# Autodesk Inventor assembly: bellows_latest
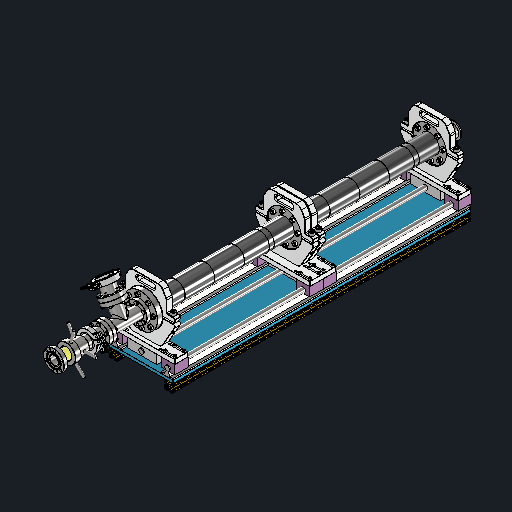
[picture p0: Inventor's stored thumbnail of the model, 512x512]
Saved by Autodesk Inventor 2027.1 (Build 311270010, 270A)
## iProperties
Created: 2026-06-04
Part Number: bellows_latest
Document SubType Name: Assembly
Designer: shusu
Author: shusu
## Documents named in this file (20)
- C:\Users\queezz\Dropbox\Drawings\pihti-cad\bellows-probe\sliding-assembly.iam
- C:\Users\queezz\Dropbox\Drawings\pihti-cad\bellows-probe\rail bwllows probe.ipt
- C:\Users\queezz\Dropbox\Drawings\pihti-cad\bellows-probe\Al-profile-30x30-L1000.ipt
- C:\Users\queezz\Dropbox\Drawings\pihti-cad\ContentCenter\Aluminium-profiles\Al-profile-30x30.ipt
- C:\Users\queezz\Dropbox\Drawings\pihti-cad\bellows-probe\base-plate-for-bellows.ipt
- C:\Users\queezz\Dropbox\Drawings\pihti-cad\ContentCenter\Fastners\M6x16-SHCS.ipt
- C:\Users\queezz\Dropbox\Drawings\pihti-cad\ContentCenter\CF-KF-adapters\ICF70_to_KF40.ipt
- C:\Users\queezz\Dropbox\Drawings\pihti-cad\bellows-probe\CF114-CF70-zero-length-adappter.ipt
- C:\Users\queezz\Dropbox\Drawings\pihti-cad\bellows-probe\M16-lead-screw.ipt
- C:\Users\queezz\Dropbox\Drawings\pihti-cad\bellows-probe\lead-screw-nut-preview.ipt
- C:\Users\queezz\Dropbox\Drawings\pihti-cad\bellows-probe\two-section-bellows-on-bearings.iam
- C:\Users\queezz\Dropbox\Drawings\pihti-cad\ContentCenter\Fastners\m8-nut.ipt
- C:\Users\queezz\Dropbox\Drawings\pihti-cad\ContentCenter\Fastners\M8x45-HexCS.ipt
- C:\Users\queezz\Dropbox\Drawings\pihti-cad\bellows-probe\mizuno-pipe.iam
- C:\Users\queezz\Dropbox\Drawings\pihti-cad\Plasma Vessel\pipe-o-ring-gauge-port-assembly.iam
- C:\Users\queezz\Dropbox\Drawings\pihti-cad\ContentCenter\CF-parts\CF-70-Tee.ipt
- C:\Users\queezz\Dropbox\Drawings\pihti-cad\ContentCenter\Fastners\M6x25-HexCS.ipt
- C:\Users\queezz\Dropbox\Drawings\pihti-cad\ContentCenter\Fastners\M6x35-HexCS.ipt
- C:\Users\queezz\Dropbox\Drawings\pihti-cad\ContentCenter\Fastners\M6-nut.ipt
- C:\Users\queezz\Dropbox\Drawings\pihti-cad\ContentCenter\NW\NW40_clamp.ipt
## Components (82 placed, 45 different names)
1. rail:1 — Mate:9, Flush:22, Mate:30
2. rail:2 — Mate:9, Mate:16, Flush:12, Flush:20
3. Al-profile-30x30-L1000:1 — Mate:18, Flush:13, Flush:16
4. Al-profile-30x30-L1000:2 — Mate:17, Flush:14, Flush:15
5. base-plate-for-bellows:1 — Mate:16, Flush:11, Flush:12, Mate:17, Mate:18, Flush:13, Flush:14, Flush:15, Flush:16, Flush:22, Mate:30, Flush:24
6. ICF70_to_KF40:1 — Rotational:6, Mate:31
7. CF114-CF70-zero-length-adappter:1 — Rotational:6, Rear flange bolt 1 - rigid, Rear flange bolt 2 - rigid, Rear flange bolt 3 - rigid, Rear flange bolt 4 - rigid, Rear flange bolt 5 - rigid, Rear flange bolt 6 - rigid, Rear flange bolt 7 - rigid, Rear flange bolt 8 - rigid
8. M16-lead-screw:1 — Mate:26, Flush:20
9. lead-screw-nut-preview:1 — Mate:26, Rigid:25
10. lead-screw-nut-preview:2
11. lead-screw-nut-preview:4
12. two-section-bellows-on-bearings:1 [sub-assembly] — Rigid:25, Rigid:26, Front flange nut 1 - rigid, Rear flange nut 1 - rigid, Front flange nut 2 - rigid, Front flange nut 3 - rigid, Front flange nut 4 - rigid, Front flange nut 5 - rigid, Front flange nut 6 - rigid, Front flange nut 7 - rigid, Front flange nut 8 - rigid, Rear flange nut 2 - rigid, Rear flange nut 3 - rigid, Rear flange nut 4 - rigid, Rear flange nut 5 - rigid, Rear flange nut 6 - rigid, Rear flange nut 7 - rigid, Rear flange nut 8 - rigid, Flush:24
13. CF114-CF70-zero-length-adappter:2 — Rigid:26, Front flange bolt 1 - rigid, Front flange bolt 2 - rigid, Front flange bolt 3 - rigid, Front flange bolt 4 - rigid, Front flange bolt 5 - rigid, Front flange bolt 6 - rigid, Front flange bolt 7 - rigid, Front flange bolt 8 - rigid, Rigid:60, Flush:23, Bypass tee to bellows adapter - rigid
14. mizuno-pipe:1 [sub-assembly] — Mate:31, Flush:23
15. pipe-o-ring-gauge-port-assembly:1 [sub-assembly] — Rigid:60, Gauge port to bypass tee - rigid, Bypass gauge nut 1 - rigid, Bypass gauge nut 2 - rigid, Bypass gauge nut 3 - rigid, Bypass gauge nut 4 - rigid, Bypass gauge nut 5 - rigid, Bypass gauge nut 6 - rigid
16. CF-70-Tee:1 — Bypass tee to bellows adapter - rigid, Gauge port to bypass tee - rigid, Bypass bellows bolt 1 - rigid, Bypass bellows bolt 2 - rigid, Bypass bellows bolt 3 - rigid, Bypass bellows bolt 4 - rigid, Bypass bellows bolt 5 - rigid, Bypass bellows bolt 6 - rigid, Bypass gauge bolt 1 - rigid, Bypass gauge bolt 2 - rigid, Bypass gauge bolt 3 - rigid, Bypass gauge bolt 4 - rigid, Bypass gauge bolt 5 - rigid, Bypass gauge bolt 6 - rigid, Rigid:81, Bypass branch bolt 1 - rigid, Bypass branch bolt 2 - rigid, Bypass branch bolt 3 - rigid, Bypass branch bolt 4 - rigid, Bypass branch bolt 5 - rigid, Bypass branch bolt 6 - rigid
17. ICF70_to_KF40:2 — Rigid:81, Bypass branch nut 1 - rigid, Bypass branch nut 2 - rigid, Bypass branch nut 3 - rigid, Bypass branch nut 4 - rigid, Bypass branch nut 5 - rigid, Bypass branch nut 6 - rigid, Bypass KF40 clamp to adapter - rigid
18. Bypass branch bolt 1 — Bypass branch bolt 1 - rigid
19. Bypass branch nut 1 — Bypass branch nut 1 - rigid
20. Bypass branch bolt 2 — Bypass branch bolt 2 - rigid
21. Bypass branch nut 2 — Bypass branch nut 2 - rigid
22. Bypass branch bolt 3 — Bypass branch bolt 3 - rigid
23. Bypass branch nut 3 — Bypass branch nut 3 - rigid
24. Bypass branch bolt 4 — Bypass branch bolt 4 - rigid
25. Bypass branch nut 4 — Bypass branch nut 4 - rigid
26. Bypass branch bolt 5 — Bypass branch bolt 5 - rigid
27. Bypass branch nut 5 — Bypass branch nut 5 - rigid
28. Bypass branch bolt 6 — Bypass branch bolt 6 - rigid
29. Bypass branch nut 6 — Bypass branch nut 6 - rigid
30. Bypass branch KF40 clamp:1 — Bypass KF40 clamp to adapter - rigid
31. Bypass bellows bolt 1 — Bypass bellows bolt 1 - rigid
32. Bypass bellows bolt 2 — Bypass bellows bolt 2 - rigid
33. Bypass bellows bolt 3 — Bypass bellows bolt 3 - rigid
34. Bypass bellows bolt 4 — Bypass bellows bolt 4 - rigid
35. Bypass bellows bolt 5 — Bypass bellows bolt 5 - rigid
36. Bypass bellows bolt 6 — Bypass bellows bolt 6 - rigid
37. Bypass gauge bolt 1 — Bypass gauge bolt 1 - rigid
38. Bypass gauge nut 1 — Bypass gauge nut 1 - rigid
39. Bypass gauge bolt 2 — Bypass gauge bolt 2 - rigid
40. Bypass gauge nut 2 — Bypass gauge nut 2 - rigid
41. Bypass gauge bolt 3 — Bypass gauge bolt 3 - rigid
42. Bypass gauge nut 3 — Bypass gauge nut 3 - rigid
43. Bypass gauge bolt 4 — Bypass gauge bolt 4 - rigid
44. Bypass gauge nut 4 — Bypass gauge nut 4 - rigid
45. Bypass gauge bolt 5 — Bypass gauge bolt 5 - rigid
46. Bypass gauge nut 5 — Bypass gauge nut 5 - rigid
47. Bypass gauge bolt 6 — Bypass gauge bolt 6 - rigid
48. Bypass gauge nut 6 — Bypass gauge nut 6 - rigid
49. AS 1112 (2) - Metric M8  Type 5:1 — Front flange nut 1 - rigid
50. AS 1427 - Metric M8 x 45:1 — Front flange bolt 1 - rigid
51. AS 1427 - Metric M8 x 45:2 — Rear flange bolt 1 - rigid
52. AS 1112 (2) - Metric M8  Type 5:2 — Rear flange nut 1 - rigid
53. AS 1427 - Metric M8 x 45:3 — Front flange bolt 2 - rigid
54. AS 1427 - Metric M8 x 45:4 — Front flange bolt 3 - rigid
55. AS 1427 - Metric M8 x 45:5 — Front flange bolt 4 - rigid
56. AS 1427 - Metric M8 x 45:6 — Front flange bolt 5 - rigid
57. AS 1427 - Metric M8 x 45:7 — Front flange bolt 6 - rigid
58. AS 1427 - Metric M8 x 45:8 — Front flange bolt 7 - rigid
59. AS 1427 - Metric M8 x 45:9 — Front flange bolt 8 - rigid
60. AS 1427 - Metric M8 x 45:10 — Rear flange bolt 2 - rigid
61. AS 1427 - Metric M8 x 45:11 — Rear flange bolt 3 - rigid
62. AS 1427 - Metric M8 x 45:12 — Rear flange bolt 4 - rigid
63. AS 1427 - Metric M8 x 45:13 — Rear flange bolt 5 - rigid
64. AS 1427 - Metric M8 x 45:14 — Rear flange bolt 6 - rigid
65. AS 1427 - Metric M8 x 45:15 — Rear flange bolt 7 - rigid
66. AS 1427 - Metric M8 x 45:16 — Rear flange bolt 8 - rigid
67. AS 1112 (2) - Metric M8  Type 5:3 — Front flange nut 2 - rigid
68. AS 1112 (2) - Metric M8  Type 5:4 — Front flange nut 3 - rigid
69. AS 1112 (2) - Metric M8  Type 5:5 — Front flange nut 4 - rigid
70. AS 1112 (2) - Metric M8  Type 5:6 — Front flange nut 5 - rigid
71. AS 1112 (2) - Metric M8  Type 5:7 — Front flange nut 6 - rigid
72. AS 1112 (2) - Metric M8  Type 5:8 — Front flange nut 7 - rigid
73. AS 1112 (2) - Metric M8  Type 5:9 — Front flange nut 8 - rigid
74. AS 1112 (2) - Metric M8  Type 5:10 — Rear flange nut 2 - rigid
75. AS 1112 (2) - Metric M8  Type 5:11 — Rear flange nut 3 - rigid
76. AS 1112 (2) - Metric M8  Type 5:12 — Rear flange nut 4 - rigid
77. AS 1112 (2) - Metric M8  Type 5:13 — Rear flange nut 5 - rigid
78. AS 1112 (2) - Metric M8  Type 5:14 — Rear flange nut 6 - rigid
79. AS 1112 (2) - Metric M8  Type 5:15 — Rear flange nut 7 - rigid
80. AS 1112 (2) - Metric M8  Type 5:16 — Rear flange nut 8 - rigid
81. JIS B 1176 - Metric M6 x 16:3
82. JIS B 1176 - Metric M6 x 16:4
## Relationships (100: WeldJoint 74, Mate 15, Flush 10, RevoluteJoint 1)
- [Mate]: rail:1 ↔ two-section-bellows-on-bearings:1
- [Mate]: rail:2 ↔ two-section-bellows-on-bearings:1
- [Mate]: rail:2 ↔ two-section-bellows-on-bearings:1
- [Mate]: rail:1 ↔ two-section-bellows-on-bearings:1
- Mate:9 (175 mm): rail:1 ↔ rail:2
- [Mate]: two-section-bellows-on-bearings:1
- [Mate]: two-section-bellows-on-bearings:1
- Mate:16: rail:2 ↔ base-plate-for-bellows:1
- Flush:11: base-plate-for-bellows:1
- Flush:12: rail:2 ↔ base-plate-for-bellows:1
- Mate:17: Al-profile-30x30-L1000:2 ↔ base-plate-for-bellows:1
- Mate:18: Al-profile-30x30-L1000:1 ↔ base-plate-for-bellows:1
- Flush:13: Al-profile-30x30-L1000:1 ↔ base-plate-for-bellows:1
- Flush:14: Al-profile-30x30-L1000:2 ↔ base-plate-for-bellows:1
- Flush:15: Al-profile-30x30-L1000:2 ↔ base-plate-for-bellows:1
- Flush:16: Al-profile-30x30-L1000:1 ↔ base-plate-for-bellows:1
- [WeldJoint]: two-section-bellows-on-bearings:1 ↔ JIS B 1176 - Metric M6 x 16:3
- [WeldJoint]: two-section-bellows-on-bearings:1 ↔ JIS B 1176 - Metric M6 x 16:4
- [WeldJoint]: CF114-CF70-zero-length-adappter:1 ↔ two-section-bellows-on-bearings:1
- Rotational:6 [RevoluteJoint]: ICF70_to_KF40:1 ↔ CF114-CF70-zero-length-adappter:1
- Mate:26: M16-lead-screw:1 ↔ lead-screw-nut-preview:1
- Flush:20: rail:2 ↔ M16-lead-screw:1
- [WeldJoint]: lead-screw-nut-preview:2 ↔ two-section-bellows-on-bearings:1
- [Mate]: rail:1 ↔ two-section-bellows-on-bearings:1
- [Mate]: rail:2 ↔ two-section-bellows-on-bearings:1
- [WeldJoint]: lead-screw-nut-preview:4 ↔ two-section-bellows-on-bearings:1
- Rigid:25 [WeldJoint]: lead-screw-nut-preview:1 ↔ two-section-bellows-on-bearings:1
- Rigid:26 [WeldJoint]: two-section-bellows-on-bearings:1 ↔ CF114-CF70-zero-length-adappter:2
- Front flange nut 1 - rigid [WeldJoint]: two-section-bellows-on-bearings:1 ↔ AS 1112 (2) - Metric M8  Type 5:1
- Front flange bolt 1 - rigid [WeldJoint]: CF114-CF70-zero-length-adappter:2 ↔ AS 1427 - Metric M8 x 45:1
- Rear flange bolt 1 - rigid [WeldJoint]: CF114-CF70-zero-length-adappter:1 ↔ AS 1427 - Metric M8 x 45:2
- Rear flange nut 1 - rigid [WeldJoint]: two-section-bellows-on-bearings:1 ↔ AS 1112 (2) - Metric M8  Type 5:2
- Front flange bolt 2 - rigid [WeldJoint]: CF114-CF70-zero-length-adappter:2 ↔ AS 1427 - Metric M8 x 45:3
- Front flange nut 2 - rigid [WeldJoint]: two-section-bellows-on-bearings:1 ↔ AS 1112 (2) - Metric M8  Type 5:3
- Front flange bolt 3 - rigid [WeldJoint]: CF114-CF70-zero-length-adappter:2 ↔ AS 1427 - Metric M8 x 45:4
- Front flange nut 3 - rigid [WeldJoint]: two-section-bellows-on-bearings:1 ↔ AS 1112 (2) - Metric M8  Type 5:4
- Front flange bolt 4 - rigid [WeldJoint]: CF114-CF70-zero-length-adappter:2 ↔ AS 1427 - Metric M8 x 45:5
- Front flange nut 4 - rigid [WeldJoint]: two-section-bellows-on-bearings:1 ↔ AS 1112 (2) - Metric M8  Type 5:5
- Front flange bolt 5 - rigid [WeldJoint]: CF114-CF70-zero-length-adappter:2 ↔ AS 1427 - Metric M8 x 45:6
- Front flange nut 5 - rigid [WeldJoint]: two-section-bellows-on-bearings:1 ↔ AS 1112 (2) - Metric M8  Type 5:6
- Front flange bolt 6 - rigid [WeldJoint]: CF114-CF70-zero-length-adappter:2 ↔ AS 1427 - Metric M8 x 45:7
- Front flange nut 6 - rigid [WeldJoint]: two-section-bellows-on-bearings:1 ↔ AS 1112 (2) - Metric M8  Type 5:7
- Front flange bolt 7 - rigid [WeldJoint]: CF114-CF70-zero-length-adappter:2 ↔ AS 1427 - Metric M8 x 45:8
- Front flange nut 7 - rigid [WeldJoint]: two-section-bellows-on-bearings:1 ↔ AS 1112 (2) - Metric M8  Type 5:8
- Front flange bolt 8 - rigid [WeldJoint]: CF114-CF70-zero-length-adappter:2 ↔ AS 1427 - Metric M8 x 45:9
- Front flange nut 8 - rigid [WeldJoint]: two-section-bellows-on-bearings:1 ↔ AS 1112 (2) - Metric M8  Type 5:9
- Rear flange bolt 2 - rigid [WeldJoint]: CF114-CF70-zero-length-adappter:1 ↔ AS 1427 - Metric M8 x 45:10
- Rear flange nut 2 - rigid [WeldJoint]: two-section-bellows-on-bearings:1 ↔ AS 1112 (2) - Metric M8  Type 5:10
- Rear flange bolt 3 - rigid [WeldJoint]: CF114-CF70-zero-length-adappter:1 ↔ AS 1427 - Metric M8 x 45:11
- Rear flange nut 3 - rigid [WeldJoint]: two-section-bellows-on-bearings:1 ↔ AS 1112 (2) - Metric M8  Type 5:11
- Rear flange bolt 4 - rigid [WeldJoint]: CF114-CF70-zero-length-adappter:1 ↔ AS 1427 - Metric M8 x 45:12
- Rear flange nut 4 - rigid [WeldJoint]: two-section-bellows-on-bearings:1 ↔ AS 1112 (2) - Metric M8  Type 5:12
- Rear flange bolt 5 - rigid [WeldJoint]: CF114-CF70-zero-length-adappter:1 ↔ AS 1427 - Metric M8 x 45:13
- Rear flange nut 5 - rigid [WeldJoint]: two-section-bellows-on-bearings:1 ↔ AS 1112 (2) - Metric M8  Type 5:13
- Rear flange bolt 6 - rigid [WeldJoint]: CF114-CF70-zero-length-adappter:1 ↔ AS 1427 - Metric M8 x 45:14
- Rear flange nut 6 - rigid [WeldJoint]: two-section-bellows-on-bearings:1 ↔ AS 1112 (2) - Metric M8  Type 5:14
- Rear flange bolt 7 - rigid [WeldJoint]: CF114-CF70-zero-length-adappter:1 ↔ AS 1427 - Metric M8 x 45:15
- Rear flange nut 7 - rigid [WeldJoint]: two-section-bellows-on-bearings:1 ↔ AS 1112 (2) - Metric M8  Type 5:15
- Rear flange bolt 8 - rigid [WeldJoint]: CF114-CF70-zero-length-adappter:1 ↔ AS 1427 - Metric M8 x 45:16
- Rear flange nut 8 - rigid [WeldJoint]: two-section-bellows-on-bearings:1 ↔ AS 1112 (2) - Metric M8  Type 5:16
- Flush:22: rail:1 ↔ base-plate-for-bellows:1
- Mate:30: rail:1 ↔ base-plate-for-bellows:1
- Rigid:60 [WeldJoint]: CF114-CF70-zero-length-adappter:2 ↔ pipe-o-ring-gauge-port-assembly:1
- Mate:31: ICF70_to_KF40:1 ↔ mizuno-pipe:1
- Flush:23 (-290 mm): CF114-CF70-zero-length-adappter:2 ↔ mizuno-pipe:1
- Flush:24: base-plate-for-bellows:1 ↔ two-section-bellows-on-bearings:1
- Bypass tee to bellows adapter - rigid [WeldJoint]: CF114-CF70-zero-length-adappter:2 ↔ CF-70-Tee:1
- Gauge port to bypass tee - rigid [WeldJoint]: pipe-o-ring-gauge-port-assembly:1 ↔ CF-70-Tee:1
- Bypass bellows bolt 1 - rigid [WeldJoint]: CF-70-Tee:1 ↔ Bypass bellows bolt 1
- Bypass bellows bolt 2 - rigid [WeldJoint]: CF-70-Tee:1 ↔ Bypass bellows bolt 2
- Bypass bellows bolt 3 - rigid [WeldJoint]: CF-70-Tee:1 ↔ Bypass bellows bolt 3
- Bypass bellows bolt 4 - rigid [WeldJoint]: CF-70-Tee:1 ↔ Bypass bellows bolt 4
- Bypass bellows bolt 5 - rigid [WeldJoint]: CF-70-Tee:1 ↔ Bypass bellows bolt 5
- Bypass bellows bolt 6 - rigid [WeldJoint]: CF-70-Tee:1 ↔ Bypass bellows bolt 6
- Bypass gauge bolt 1 - rigid [WeldJoint]: CF-70-Tee:1 ↔ Bypass gauge bolt 1
- Bypass gauge nut 1 - rigid [WeldJoint]: pipe-o-ring-gauge-port-assembly:1 ↔ Bypass gauge nut 1
- Bypass gauge bolt 2 - rigid [WeldJoint]: CF-70-Tee:1 ↔ Bypass gauge bolt 2
- Bypass gauge nut 2 - rigid [WeldJoint]: pipe-o-ring-gauge-port-assembly:1 ↔ Bypass gauge nut 2
- Bypass gauge bolt 3 - rigid [WeldJoint]: CF-70-Tee:1 ↔ Bypass gauge bolt 3
- Bypass gauge nut 3 - rigid [WeldJoint]: pipe-o-ring-gauge-port-assembly:1 ↔ Bypass gauge nut 3
- Bypass gauge bolt 4 - rigid [WeldJoint]: CF-70-Tee:1 ↔ Bypass gauge bolt 4
- Bypass gauge nut 4 - rigid [WeldJoint]: pipe-o-ring-gauge-port-assembly:1 ↔ Bypass gauge nut 4
- Bypass gauge bolt 5 - rigid [WeldJoint]: CF-70-Tee:1 ↔ Bypass gauge bolt 5
- Bypass gauge nut 5 - rigid [WeldJoint]: pipe-o-ring-gauge-port-assembly:1 ↔ Bypass gauge nut 5
- Bypass gauge bolt 6 - rigid [WeldJoint]: CF-70-Tee:1 ↔ Bypass gauge bolt 6
- Bypass gauge nut 6 - rigid [WeldJoint]: pipe-o-ring-gauge-port-assembly:1 ↔ Bypass gauge nut 6
- Rigid:81 [WeldJoint]: CF-70-Tee:1 ↔ ICF70_to_KF40:2
- Bypass branch bolt 1 - rigid [WeldJoint]: CF-70-Tee:1 ↔ Bypass branch bolt 1
- Bypass branch nut 1 - rigid [WeldJoint]: ICF70_to_KF40:2 ↔ Bypass branch nut 1
- Bypass branch bolt 2 - rigid [WeldJoint]: CF-70-Tee:1 ↔ Bypass branch bolt 2
- Bypass branch nut 2 - rigid [WeldJoint]: ICF70_to_KF40:2 ↔ Bypass branch nut 2
- Bypass branch bolt 3 - rigid [WeldJoint]: CF-70-Tee:1 ↔ Bypass branch bolt 3
- Bypass branch nut 3 - rigid [WeldJoint]: ICF70_to_KF40:2 ↔ Bypass branch nut 3
- Bypass branch bolt 4 - rigid [WeldJoint]: CF-70-Tee:1 ↔ Bypass branch bolt 4
- Bypass branch nut 4 - rigid [WeldJoint]: ICF70_to_KF40:2 ↔ Bypass branch nut 4
- Bypass branch bolt 5 - rigid [WeldJoint]: CF-70-Tee:1 ↔ Bypass branch bolt 5
- Bypass branch nut 5 - rigid [WeldJoint]: ICF70_to_KF40:2 ↔ Bypass branch nut 5
- Bypass branch bolt 6 - rigid [WeldJoint]: CF-70-Tee:1 ↔ Bypass branch bolt 6
- Bypass branch nut 6 - rigid [WeldJoint]: ICF70_to_KF40:2 ↔ Bypass branch nut 6
- Bypass KF40 clamp to adapter - rigid [WeldJoint] (-6.095 mm): ICF70_to_KF40:2 ↔ Bypass branch KF40 clamp:1
